# Autodesk Inventor assembly: With Flush Mount Spacer
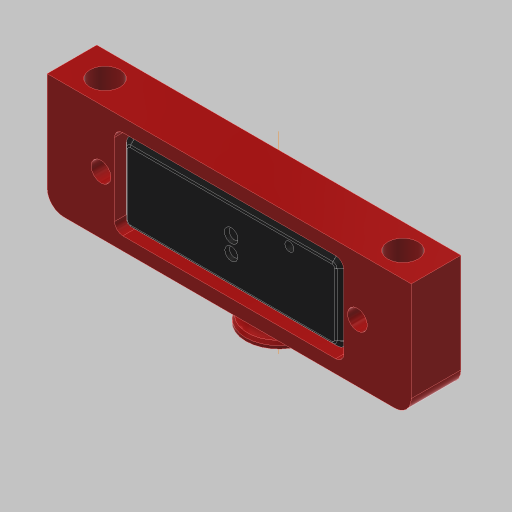
[picture p0: Inventor's stored thumbnail of the model, 512x512]
Saved by Autodesk Inventor 2023.5 (Build 275446000, 446)
## iProperties
Created: 2025-02-08
Part Number: With Flush Mount Spacer
Document SubType Name: Assembly
Designer: slick
Author: slick
## Documents named in this file (3)
- C:\Users\slick\OneDrive\Desktop\2025-ReefScape---CAD\STEP files\sen36005_3d_model\With Flush Mount Spacer.iam
- C:\Users\slick\OneDrive\Desktop\2025-ReefScape---CAD\STEP files\sen36005_3d_model\sen36005_3d_model.iam
- C:\Users\slick\OneDrive\Desktop\2025-ReefScape---CAD\STEP files\sen36005_3d_model\Spacer.ipt
## Components (2 placed, 2 different names)
1. sen36005_3d_model:1 [sub-assembly] — Insert:1, Insert:2
2. Spacer:1 — Insert:1, Insert:2
## Relationships (2: Insert 2)
- Insert:1: sen36005_3d_model:1 ↔ Spacer:1
- Insert:2: sen36005_3d_model:1 ↔ Spacer:1
